# Autodesk Inventor assembly: finalBox
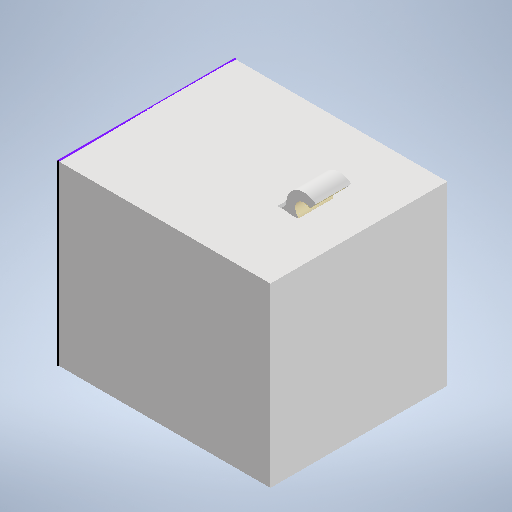
[picture p0: Inventor's stored thumbnail of the model, 512x512]
Saved by Autodesk Inventor 2025.2 (Build 292293000, 293)
## iProperties
Created: 2025-02-04
Part Number: finalBox
Document SubType Name: Assembly
Designer: sujay
Author: sujay
## Documents named in this file (4)
- C:\Users\sujay\OneDrive\Documents\Inventor\HUNCH\finalBox.iam
- C:\Users\sujay\OneDrive\Documents\Inventor\HUNCH\box-1.ipt
- C:\Users\sujay\OneDrive\Documents\Inventor\HUNCH\door.ipt
- C:\Users\sujay\OneDrive\Documents\Inventor\HUNCH\pushingThingy.ipt
## Components (3 placed, 3 different names)
1. box-1:1 — Rotational:1, Rotational:2
2. door:1 — Rotational:1
3. pushingThingy:1 — Rotational:2
## Relationships (2: RevoluteJoint 2)
- Rotational:1 [RevoluteJoint]: box-1:1 ↔ door:1
- Rotational:2 [RevoluteJoint]: box-1:1 ↔ pushingThingy:1
